# Autodesk Inventor assembly: Cart main body
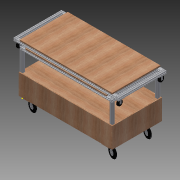
[picture p0: Inventor's stored thumbnail of the model, 180x180]
Saved by Autodesk Inventor 2013 (Build 170138000, 138)
## iProperties
Created: 2013-01-03
Part Number: Cart main body
Document SubType Name: Assembly
Designer: Arpan
Author: Arpan
## Documents named in this file (11)
- C:\Users\Arpan\Documents\GitHub\frc2013CAD\Cart- Take 2\Cart main body.iam
- C:\Users\Arpan\Documents\GitHub\frc2013CAD\Cart- Take 2\28 piece.ipt
- C:\Users\Arpan\Documents\GitHub\frc2013CAD\Cart- Take 2\49 piece.ipt
- C:\Users\Arpan\Documents\GitHub\frc2013CAD\Cart- Take 2\Wheel mount plate.ipt
- C:\Users\Arpan\Documents\GitHub\frc2013CAD\Cart- Take 2\20.75 piece.ipt
- C:\Users\Arpan\Documents\GitHub\frc2013CAD\Cart- Take 2\cart top.ipt
- C:\Users\Arpan\Documents\GitHub\frc2013CAD\Cart- Take 2\cart shelf.ipt
- C:\Users\Arpan\Documents\GitHub\frc2013CAD\Cart- Take 2\pneumatic caster\caster.iam
- C:\Users\Arpan\Documents\GitHub\frc2013CAD\Cart- Take 2\side.ipt
- C:\Users\Arpan\Documents\GitHub\frc2013CAD\Cart- Take 2\cart front.ipt
- C:\Users\Arpan\Documents\GitHub\frc2013CAD\Cart- Take 2\saddle cart.iam
## Components (27 placed, 10 different names)
1. 28 piece:1 — Mate:1, Flush:1, Flush:2, Mate:2, Flush:3, Flush:4, Mate:6, Mate:7, Mate:8, Flush:13, Flush:14, Mate:9, Flush:15, Flush:16, Mate:17, Flush:31
2. 28 piece:2 — Mate:3, Flush:5, Flush:6, Flush:7, Flush:8, Mate:5, Mate:10, Flush:17, Flush:18, Mate:11, Flush:19, Flush:20
3. 49 piece:1 — Mate:1, Flush:1, Flush:2, Flush:7, Flush:8, Flush:10, Flush:11
4. 49 piece:2 — Mate:2, Flush:3, Flush:4, Mate:3, Flush:5, Flush:6, Mate:4, Flush:9, Flush:12, Flush:32
5. Wheel mount plate:1 — Mate:4, Flush:9, Flush:10, Mate:5, Mate:24, Flush:37, Flush:38, Mate:25, Flush:39, Flush:40
6. Wheel mount plate:2 — Flush:11, Flush:12, Mate:6, Mate:7, Mate:26, Mate:27, Flush:41, Flush:42, Flush:43, Flush:44
7. 20.75 piece:1 — Mate:10, Flush:17, Flush:18, Flush:36
8. 20.75 piece:2 — Mate:11, Flush:19, Flush:20, Mate:13, Flush:23, Flush:24, Flush:33, Flush:35
9. 20.75 piece:3 — Mate:9, Flush:15, Flush:16, Mate:12, Flush:21, Flush:22, Mate:18, Mate:20, Flush:34, Flush:45
10. 20.75 piece:4 — Mate:8, Flush:13, Flush:14, Mate:19, Flush:48
11. 49 piece:3 — Mate:14, Flush:25, Flush:26, Mate:16, Flush:30, Mate:21
12. 49 piece:4 — Mate:15, Flush:27, Flush:28, Mate:22
13. 28 piece:3 — Mate:12, Flush:21, Flush:22, Mate:14, Flush:25, Flush:26, Flush:29
14. 28 piece:4 — Mate:13, Flush:23, Flush:24, Mate:15, Flush:27, Flush:28, Mate:31, Mate:32
15. cart top:1 — Mate:16, Flush:29, Flush:30, Flush:51, Flush:52, Mate:32
16. cart shelf:1 — Mate:17, Flush:31, Flush:32
17. 49 piece:5 — Mate:18, Mate:20, Flush:34, Mate:21
18. 49 piece:6 — Mate:19, Flush:33, Mate:22, Mate:23
19. cart shelf:2 — Mate:23, Flush:35, Flush:36, Mate:28, Flush:46, Mate:29, Flush:47, Mate:30, Flush:49
20. caster:1 [sub-assembly] — Mate:26, Flush:41, Flush:43
21. caster:2 [sub-assembly] — Mate:25, Flush:39, Flush:40
22. caster:3 [sub-assembly] — Mate:24, Flush:37, Flush:38
23. caster:4 [sub-assembly] — Mate:27, Flush:42, Flush:44
24. side:1 — Mate:28, Flush:45, Flush:46, Flush:50
25. side:2 — Mate:29, Flush:47, Flush:48
26. cart front:1 — Mate:30, Flush:49, Flush:50
27. saddle cart:1 [sub-assembly] — Mate:31, Flush:51, Flush:52
## Relationships (84: Flush 52, Mate 32)
- Mate:1: 28 piece:1 ↔ 49 piece:1
- Flush:1: 28 piece:1 ↔ 49 piece:1
- Flush:2: 28 piece:1 ↔ 49 piece:1
- Mate:2: 28 piece:1 ↔ 49 piece:2
- Flush:3: 28 piece:1 ↔ 49 piece:2
- Flush:4: 28 piece:1 ↔ 49 piece:2
- Mate:3: 28 piece:2 ↔ 49 piece:2
- Flush:5: 28 piece:2 ↔ 49 piece:2
- Flush:6: 28 piece:2 ↔ 49 piece:2
- Flush:7: 28 piece:2 ↔ 49 piece:1
- Flush:8: 28 piece:2 ↔ 49 piece:1
- Mate:4: 49 piece:2 ↔ Wheel mount plate:1
- Flush:9: 49 piece:2 ↔ Wheel mount plate:1
- Flush:10: 49 piece:1 ↔ Wheel mount plate:1
- Mate:5: 28 piece:2 ↔ Wheel mount plate:1
- Flush:11: 49 piece:1 ↔ Wheel mount plate:2
- Flush:12: 49 piece:2 ↔ Wheel mount plate:2
- Mate:6: 28 piece:1 ↔ Wheel mount plate:2
- Mate:7: 28 piece:1 ↔ Wheel mount plate:2
- Mate:8: 28 piece:1 ↔ 20.75 piece:4
- Flush:13: 28 piece:1 ↔ 20.75 piece:4
- Flush:14: 28 piece:1 ↔ 20.75 piece:4
- Mate:9: 28 piece:1 ↔ 20.75 piece:3
- Flush:15: 28 piece:1 ↔ 20.75 piece:3
- Flush:16: 28 piece:1 ↔ 20.75 piece:3
- Mate:10: 28 piece:2 ↔ 20.75 piece:1
- Flush:17: 28 piece:2 ↔ 20.75 piece:1
- Flush:18: 28 piece:2 ↔ 20.75 piece:1
- Mate:11: 28 piece:2 ↔ 20.75 piece:2
- Flush:19: 28 piece:2 ↔ 20.75 piece:2
- Flush:20: 28 piece:2 ↔ 20.75 piece:2
- Mate:12: 20.75 piece:3 ↔ 28 piece:3
- Flush:21: 20.75 piece:3 ↔ 28 piece:3
- Flush:22: 20.75 piece:3 ↔ 28 piece:3
- Mate:13: 20.75 piece:2 ↔ 28 piece:4
- Flush:23: 20.75 piece:2 ↔ 28 piece:4
- Flush:24: 20.75 piece:2 ↔ 28 piece:4
- Mate:14: 49 piece:3 ↔ 28 piece:3
- Flush:25: 49 piece:3 ↔ 28 piece:3
- Flush:26: 49 piece:3 ↔ 28 piece:3
- Mate:15: 49 piece:4 ↔ 28 piece:4
- Flush:27: 49 piece:4 ↔ 28 piece:4
- Flush:28: 49 piece:4 ↔ 28 piece:4
- Mate:16: 49 piece:3 ↔ cart top:1
- Flush:29: 28 piece:3 ↔ cart top:1
- Flush:30: 49 piece:3 ↔ cart top:1
- Mate:17: 28 piece:1 ↔ cart shelf:1
- Flush:31: 28 piece:1 ↔ cart shelf:1
- Flush:32: 49 piece:2 ↔ cart shelf:1
- Mate:18: 20.75 piece:3 ↔ 49 piece:5
- Mate:19: 20.75 piece:4 ↔ 49 piece:6
- Flush:33: 20.75 piece:2 ↔ 49 piece:6
- Mate:20: 20.75 piece:3 ↔ 49 piece:5
- Flush:34: 20.75 piece:3 ↔ 49 piece:5
- Mate:21 (292.1 mm): 49 piece:3 ↔ 49 piece:5
- Mate:22 (292.1 mm): 49 piece:4 ↔ 49 piece:6
- Mate:23: 49 piece:6 ↔ cart shelf:2
- Flush:35: 20.75 piece:2 ↔ cart shelf:2
- Flush:36: 20.75 piece:1 ↔ cart shelf:2
- Mate:24: Wheel mount plate:1 ↔ caster:3
- Flush:37: Wheel mount plate:1 ↔ caster:3
- Flush:38 (38.1 mm): Wheel mount plate:1 ↔ caster:3
- Mate:25: Wheel mount plate:1 ↔ caster:2
- Flush:39 (38.1 mm): Wheel mount plate:1 ↔ caster:2
- Flush:40: Wheel mount plate:1 ↔ caster:2
- Mate:26: Wheel mount plate:2 ↔ caster:1
- Mate:27: Wheel mount plate:2 ↔ caster:4
- Flush:41: Wheel mount plate:2 ↔ caster:1
- Flush:42: Wheel mount plate:2 ↔ caster:4
- Flush:43 (38.1 mm): Wheel mount plate:2 ↔ caster:1
- Flush:44 (38.1 mm): Wheel mount plate:2 ↔ caster:4
- Mate:28: cart shelf:2 ↔ side:1
- Flush:45: 20.75 piece:3 ↔ side:1
- Flush:46: cart shelf:2 ↔ side:1
- Mate:29: cart shelf:2 ↔ side:2
- Flush:47: cart shelf:2 ↔ side:2
- Flush:48: 20.75 piece:4 ↔ side:2
- Mate:30: cart shelf:2 ↔ cart front:1
- Flush:49: cart shelf:2 ↔ cart front:1
- Flush:50: side:1 ↔ cart front:1
- Mate:31: 28 piece:4 ↔ saddle cart:1
- Flush:51: cart top:1 ↔ saddle cart:1
- Flush:52: cart top:1 ↔ saddle cart:1
- Mate:32 (41.275 mm): 28 piece:4 ↔ cart top:1
